# Autodesk Inventor assembly: Inake ASs
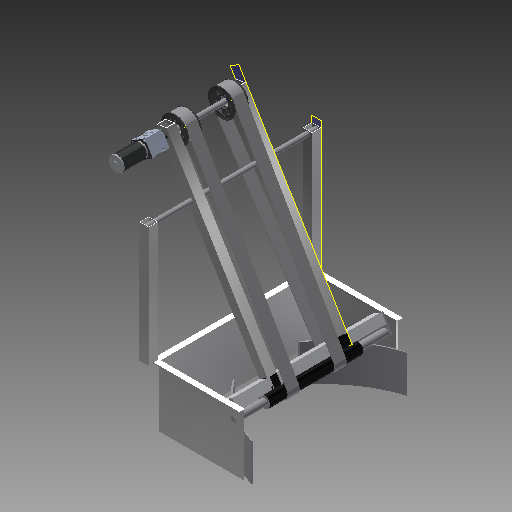
[picture p0: Inventor's stored thumbnail of the model, 512x512]
Saved by Autodesk Inventor 2017 (Build 210142000, 142)
## iProperties
Created: 2020-02-20
Part Number: Inake ASs
Document SubType Name: Assembly
Designer: S346553810
Author: S346553810
## Documents named in this file (16)
- \\ad.ocdsb.ca\studenthome\3\S338674153\FRC 2020\FullRobotRefactor\Intake\FullIntake.iam
- \\ad.ocdsb.ca\studenthome\3\S338674153\FRC 2020\FullRobotRefactor\Intake\Intake Drop.ipt
- \\ad.ocdsb.ca\studenthome\3\S338674153\FRC 2020\FullRobotRefactor\Intake\Roller cylinder.ipt
- \\ad.ocdsb.ca\studenthome\3\S338674153\FRC 2020\FullRobotRefactor\Intake\Roller Mount Piece.ipt
- \\ad.ocdsb.ca\studenthome\3\S338674153\FRC 2020\FullRobotRefactor\Intake\TexturedRoller.ipt
- \\ad.ocdsb.ca\studenthome\3\S338674153\FRC 2020\FullRobotRefactor\SubFrame\1in sq tub - 4.ipt
- \\ad.ocdsb.ca\studenthome\3\S338674153\FRC 2020\FullRobotRefactor\Intake\Kipp K0617.ipt
- \\ad.ocdsb.ca\studenthome\3\S338674153\FRC 2020\FullRobotRefactor\Intake\1in sq tub - 6-5.ipt
- \\ad.ocdsb.ca\studenthome\3\S338674153\FRC 2020\FullRobotRefactor\Intake\conveyer frame.ipt
- \\ad.ocdsb.ca\studenthome\3\S338674153\FRC 2020\FullRobotRefactor\Intake\Convery frame2.ipt
- \\ad.ocdsb.ca\studenthome\3\S338674153\FRC 2020\FullRobotRefactor\Intake\42T Wide Timing Pulley.iam
- \\ad.ocdsb.ca\studenthome\3\S338674153\FRC 2020\FullRobotRefactor\Intake\Belt.ipt
- \\ad.ocdsb.ca\studenthome\3\S338674153\FRC 2020\FullRobotRefactor\Intake\RampMount.ipt
- \\ad.ocdsb.ca\studenthome\3\S338674153\FRC 2020\FullRobotRefactor\Intake\VersaPlanetary_v1_Single_Stage_10_1_with_BAG.ipt
- \\ad.ocdsb.ca\studenthome\3\S338674153\FRC 2020\FullRobotRefactor\Intake\Part3.ipt
- \\ad.ocdsb.ca\studenthome\3\S338674153\FRC 2020\FullRobotRefactor\Intake\Funnel.ipt
## Components (22 placed, 15 different names)
1. Intake Drop:1 — Mate:1, Mate:2, Mate:3, Mate:4, Mate:6, Mate:18, Mate:19, Flush:13, Flush:14, Mate:33, Mate:34, Flush:24
2. Roller cylinder:1 — Mate:5, Mate:6, Mate:7
3. Roller Mount Piece:1 — Mate:1, Mate:2, Flush:1, Mate:5, Mate:8, Mate:9, Flush:2, Flush:3
4. Roller Mount Piece:2 — Mate:3, Mate:4, Flush:1, Flush:4, Flush:5, Mate:10
5. TexturedRoller:1 — Mate:7, Mate:8
6. 1in sq tub - 4:5 — Mate:9, Flush:2, Flush:3, Flush:7, Mate:11, Mate:25
7. 1in sq tub - 4:6 — Flush:4, Flush:5, Mate:10, Flush:6, Mate:12, Mate:13, Flush:9, Flush:15
8. Kipp K0617:6 — Mate:12, Mate:13, Mate:14, Flush:8, Mate:22
9. 1in sq tub - 6-5:1 — Mate:14, Flush:8, Flush:9, Mate:23
10. Kipp K0617:7 — Flush:6, Flush:7, Mate:11, Mate:24, Flush:16
11. Convery frame2:2 — Flush:14
12. Convery frame2:3 — Mate:18, Mate:19, Flush:13, Flush:17, Flush:18
13. conveyer frame:3 — Mate:22, Flush:15, Mate:23, Mate:26, Flush:19, Angle:2
14. conveyer frame:4 — Mate:24, Flush:16, Mate:25, Mate:30, Flush:20, Flush:21
15. RampMount:1 — Flush:17, Flush:18
16. 42T Wide Timing Pulley:1 [sub-assembly] — Mate:27, Mate:28, Mate:30, Mate:31, Mate:32
17. 42T Wide Timing Pulley:2 [sub-assembly] — Mate:28, Mate:29, Flush:22, Flush:23
18. VersaPlanetary_v1_Single_Stage_10_1_with_BAG:1 — Mate:26, Flush:19, Angle:2, Mate:27, Mate:29
19. Part3:1 — Flush:20, Flush:21
20. Belt:1 — Flush:22, Flush:23
21. Belt:2 — Mate:31, Mate:32
22. Funnel:1 — Mate:33, Mate:34, Flush:24
## Relationships (51: Mate 29, Flush 21, Angle 1)
- Mate:1: Intake Drop:1 ↔ Roller Mount Piece:1
- Mate:2: Intake Drop:1 ↔ Roller Mount Piece:1
- Mate:3: Intake Drop:1 ↔ Roller Mount Piece:2
- Mate:4: Intake Drop:1 ↔ Roller Mount Piece:2
- Flush:1: Roller Mount Piece:1 ↔ Roller Mount Piece:2
- Mate:5: Roller cylinder:1 ↔ Roller Mount Piece:1
- Mate:6: Intake Drop:1 ↔ Roller cylinder:1
- Mate:7: Roller cylinder:1 ↔ TexturedRoller:1
- Mate:8 (76.2 mm): Roller Mount Piece:1 ↔ TexturedRoller:1
- Mate:9: Roller Mount Piece:1 ↔ 1in sq tub - 4:5
- Flush:2: Roller Mount Piece:1 ↔ 1in sq tub - 4:5
- Flush:3: Roller Mount Piece:1 ↔ 1in sq tub - 4:5
- Flush:4: Roller Mount Piece:2 ↔ 1in sq tub - 4:6
- Flush:5: Roller Mount Piece:2 ↔ 1in sq tub - 4:6
- Mate:10: Roller Mount Piece:2 ↔ 1in sq tub - 4:6
- Flush:6: 1in sq tub - 4:6 ↔ Kipp K0617:7
- Flush:7: 1in sq tub - 4:5 ↔ Kipp K0617:7
- Mate:11: 1in sq tub - 4:5 ↔ Kipp K0617:7
- Mate:12: 1in sq tub - 4:6 ↔ Kipp K0617:6
- Mate:13: 1in sq tub - 4:6 ↔ Kipp K0617:6
- Mate:14: Kipp K0617:6 ↔ 1in sq tub - 6-5:1
- Flush:8: Kipp K0617:6 ↔ 1in sq tub - 6-5:1
- Flush:9: 1in sq tub - 4:6 ↔ 1in sq tub - 6-5:1
- Mate:18: Intake Drop:1 ↔ Convery frame2:3
- Mate:19: Intake Drop:1 ↔ Convery frame2:3
- Flush:13: Intake Drop:1 ↔ Convery frame2:3
- Flush:14: Intake Drop:1 ↔ Convery frame2:2
- Mate:22: Kipp K0617:6 ↔ conveyer frame:3
- Flush:15: 1in sq tub - 4:6 ↔ conveyer frame:3
- Mate:23: 1in sq tub - 6-5:1 ↔ conveyer frame:3
- Mate:24: Kipp K0617:7 ↔ conveyer frame:4
- Flush:16: Kipp K0617:7 ↔ conveyer frame:4
- Mate:25: 1in sq tub - 4:5 ↔ conveyer frame:4
- Flush:17: Convery frame2:3 ↔ RampMount:1
- Flush:18: Convery frame2:3 ↔ RampMount:1
- Mate:26: conveyer frame:3 ↔ VersaPlanetary_v1_Single_Stage_10_1_with_BAG:1
- Flush:19: conveyer frame:3 ↔ VersaPlanetary_v1_Single_Stage_10_1_with_BAG:1
- Angle:2 (90 deg): conveyer frame:3 ↔ VersaPlanetary_v1_Single_Stage_10_1_with_BAG:1
- Mate:27 (122.3518 mm): 42T Wide Timing Pulley:1 ↔ VersaPlanetary_v1_Single_Stage_10_1_with_BAG:1
- Mate:28: 42T Wide Timing Pulley:1 ↔ 42T Wide Timing Pulley:2
- Mate:29: 42T Wide Timing Pulley:2 ↔ VersaPlanetary_v1_Single_Stage_10_1_with_BAG:1
- Mate:30: conveyer frame:4 ↔ 42T Wide Timing Pulley:1
- Flush:20: conveyer frame:4 ↔ Part3:1
- Flush:21: conveyer frame:4 ↔ Part3:1
- Flush:22: 42T Wide Timing Pulley:2 ↔ Belt:1
- Flush:23: 42T Wide Timing Pulley:2 ↔ Belt:1
- Mate:31: 42T Wide Timing Pulley:1 ↔ Belt:2
- Mate:32: 42T Wide Timing Pulley:1 ↔ Belt:2
- Mate:33: Intake Drop:1 ↔ Funnel:1
- Mate:34: Intake Drop:1 ↔ Funnel:1
- Flush:24: Intake Drop:1 ↔ Funnel:1
